# Autodesk Inventor assembly: M178-PHTM-1100-01
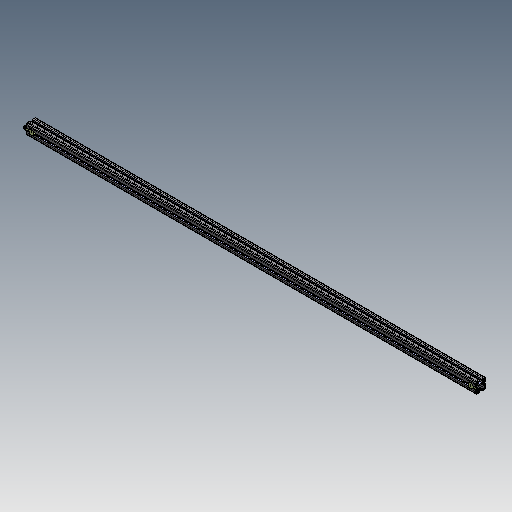
[picture p0: Inventor's stored thumbnail of the model, 512x512]
Saved by Autodesk Inventor 2018.3 (Build 223284000, 284)
## iProperties
Created: 2004-11-19
Part Number: M178-PHTM-1100-01
Document SubType Name: Assembly
Designer: Autodesk, Inc.
Manufacturer: Standard
Standards Organization: Custom
Description: PHANTOM, TABLE, TOP FRAME, CROSS BAR
Mass: 3224.27 g
Surface Area: 8325.34 cm^2
Volume: 1169.95 cm^3
Density: 2.75591 g/cm^3
CAGE: 1LJX3
Dept. ID: Product Design
Description #2: ---
Finish #1: ---
Finish #2: ---
Material ID: ---
Project Number: ---
Author: Autodesk, Inc.
## Documents named in this file (4)
- C:\AVAInvAPI\Workspace\Test Station\Components\M178-100_Cross_Phantom.iam
- C:\AVAInvAPI\Workspace\Test Station\Components\M178-1006.ipt
- C:\AVAInvAPI\Workspace\Test Station\Components\20-004.iam
- C:\Users\kelleyb.ADS\Desktop\Samples MIGRATED 2009 224 RTM_1\Standard Parts\Test Station Content\Extrusions\40 Series Profiles.ipt
## Components (3 placed, 2 different names)
1. M178-1006:1
2. 20-004:1 [sub-assembly]
3. 20-004:2 [sub-assembly]
## Relationships (4: Insert 2, Angle 2)
- [Insert]: M178-1006:1 ↔ 20-004:1
- [Angle] (0 deg): M178-1006:1 ↔ 20-004:1
- [Insert]: M178-1006:1 ↔ 20-004:2
- [Angle] (0 deg): M178-1006:1 ↔ 20-004:2
